# Autodesk Inventor assembly: chwytak_zlozenie
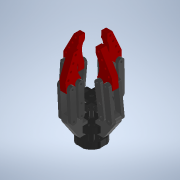
[picture p0: Inventor's stored thumbnail of the model, 180x180]
Saved by Autodesk Inventor 2022.3 (Build 263350000, 350)
## iProperties
Created: 2023-06-03
Part Number: chwytak_zlozenie
Document SubType Name: Assembly
Designer: komputer
Author: komputer
## Documents named in this file (5)
- C:\Users\komputer\Documents\Inventor\chwytak\chwytak_zlozenie.iam
- C:\Users\komputer\Documents\Inventor\chwytak\chwytak_podstawa.iam
- C:\Users\komputer\Documents\Inventor\chwytak\palec.iam
- C:\Users\komputer\Documents\Inventor\chwytak\krzyzyk.iam
- C:\Users\komputer\Documents\Inventor\chwytak\ShaftToScrewCoupler.ipt
## Components (7 placed, 4 different names)
1. chwytak_podstawa:1 [sub-assembly] — Mate:1, Mate:2, Mate:3, Mate:4, Mate:5, Mate:6, Mate:7, Mate:8, Mate:9
2. palec:1 [sub-assembly] — Mate:3, Mate:4
3. palec:2 [sub-assembly] — Mate:5, Mate:6
4. palec:3 [sub-assembly] — Mate:7, Mate:8
5. palec:4 [sub-assembly] — Mate:1, Mate:2
6. krzyzyk:1 [sub-assembly] — Mate:9, Mate:10
7. ShaftToScrewCoupler:1 — Mate:10
## Relationships (10: Mate 10)
- Mate:1 (0.5 mm): chwytak_podstawa:1 ↔ palec:4
- Mate:2: chwytak_podstawa:1 ↔ palec:4
- Mate:3 (0.5 mm): chwytak_podstawa:1 ↔ palec:1
- Mate:4: chwytak_podstawa:1 ↔ palec:1
- Mate:5 (0.5 mm): chwytak_podstawa:1 ↔ palec:2
- Mate:6: chwytak_podstawa:1 ↔ palec:2
- Mate:7 (0.5 mm): chwytak_podstawa:1 ↔ palec:3
- Mate:8: chwytak_podstawa:1 ↔ palec:3
- Mate:9: chwytak_podstawa:1 ↔ krzyzyk:1
- Mate:10: krzyzyk:1 ↔ ShaftToScrewCoupler:1
